# Autodesk Inventor assembly: Z-Holder-OneMotor
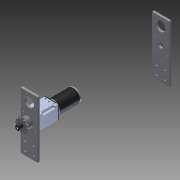
[picture p0: Inventor's stored thumbnail of the model, 180x180]
Saved by Autodesk Inventor 2013 (Build 170138000, 138)
## iProperties
Created: 2014-01-29
Part Number: Z-Holder-OneMotor
Document SubType Name: Assembly
Designer: 215152
Author: 215152
## Documents named in this file (4)
- E:\Robotics\FRC\2014\CAD\Robot\Pickup\Z-Holder-OneMotor.iam
- E:\Robotics\FRC\2014\CAD\Robot\Pickup\Z-Plate.ipt
- E:\Robotics\FRC\2014\CAD\Robot\Pickup\Imported Components\217-2 Stage Versaplanetary STEP\217-2 Stage Versaplanetary STEP.iam
- E:\Robotics\FRC\2014\CAD\Robot\Pickup\BigSprocket.ipt
## Components (4 placed, 3 different names)
1. Z-Plate:1 — Mate:1, Flush:1, Flush:2, Mate:2, Mate:3, Mate:4, Mate:5
2. Z-Plate:2 — Mate:1, Flush:1, Flush:2
3. 217-2 Stage Versaplanetary STEP:1 [sub-assembly] — Mate:2, Mate:3, Mate:4, Mate:6, Mate:7
4. BigSprocket:1 — Mate:5, Mate:6, Mate:7
## Relationships (9: Mate 7, Flush 2)
- Mate:1 (387.35 mm): Z-Plate:1 ↔ Z-Plate:2
- Flush:1: Z-Plate:1 ↔ Z-Plate:2
- Flush:2: Z-Plate:1 ↔ Z-Plate:2
- Mate:2: Z-Plate:1 ↔ 217-2 Stage Versaplanetary STEP:1
- Mate:3: Z-Plate:1 ↔ 217-2 Stage Versaplanetary STEP:1
- Mate:4: Z-Plate:1 ↔ 217-2 Stage Versaplanetary STEP:1
- Mate:5 (19.05 mm): Z-Plate:1 ↔ BigSprocket:1
- Mate:6: 217-2 Stage Versaplanetary STEP:1 ↔ BigSprocket:1
- Mate:7: 217-2 Stage Versaplanetary STEP:1 ↔ BigSprocket:1
